# Autodesk Inventor assembly: Rev Wheel
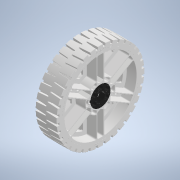
[picture p0: Inventor's stored thumbnail of the model, 180x180]
Saved by Autodesk Inventor 2022 (Build 260153000, 153)
## iProperties
Created: 2023-01-18
Part Number: Rev Wheel
Document SubType Name: Assembly
Designer: s135320
Author: s135320
## Documents named in this file (3)
- D:\Rev Wheel.iam
- D:\REV-21-2037.ipt
- D:\Traction_Wheel-6in-MAXSpline.ipt
## Components (3 placed, 2 different names)
1. REV-21-2037:1 — Mate:1, Mate:2
2. Traction_Wheel-6in-MAXSpline:1 — Mate:1, Mate:2, Mate:3, Mate:4
3. REV-21-2037:2 — Mate:3, Mate:4
## Relationships (4: Mate 4)
- Mate:1: REV-21-2037:1 ↔ Traction_Wheel-6in-MAXSpline:1
- Mate:2: REV-21-2037:1 ↔ Traction_Wheel-6in-MAXSpline:1
- Mate:3: Traction_Wheel-6in-MAXSpline:1 ↔ REV-21-2037:2
- Mate:4: Traction_Wheel-6in-MAXSpline:1 ↔ REV-21-2037:2
